# Autodesk Inventor assembly: box
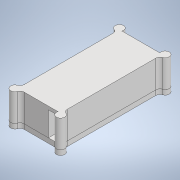
[picture p0: Inventor's stored thumbnail of the model, 180x180]
Saved by Autodesk Inventor 2020 (Build 240168000, 168)
## iProperties
Created: 2020-03-07
Part Number: box
Document SubType Name: Assembly
Designer: Richard
Author: Richard
## Documents named in this file (3)
- F:\Richard\Documents\psu\OpenZ\3d_STLs\PSU_BOX\box.iam
- F:\Richard\Documents\psu\OpenZ\3d_STLs\PSU_BOX\box.ipt
- F:\Richard\Documents\psu\OpenZ\3d_STLs\PSU_BOX\Lid.ipt
## Components (2 placed, 2 different names)
1. box:1 — Mate:1, Insert:1, Insert:2
2. Lid:1 — Mate:1, Insert:1, Insert:2
## Relationships (3: Insert 2, Mate 1)
- Mate:1: box:1 ↔ Lid:1
- Insert:1: box:1 ↔ Lid:1
- Insert:2: box:1 ↔ Lid:1
